# Autodesk Inventor assembly: HopperAssembly_v2
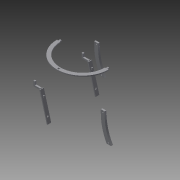
[picture p0: Inventor's stored thumbnail of the model, 180x180]
Saved by Autodesk Inventor 2013 (Build 170138000, 138)
## iProperties
Created: 2013-01-17
Part Number: HopperAssembly_v2
Document SubType Name: Assembly
Designer: twsass
Author: twsass
## Documents named in this file (5)
- E:\Robotics\Hopper\HopperAssembly_v2.iam
- E:\Robotics\Hopper\AttachmentPlateHopper_v2.ipt
- E:\Robotics\Hopper\HopperFrontSupport_v1.ipt
- E:\Robotics\Hopper\HopperSupportRod_v1.ipt
- E:\Robotics\Hopper\TopfemaleHoopSection_v1.ipt
## Components (7 placed, 4 different names)
1. AttachmentPlateHopper_v2:1 — Mate:4, Mate:5, Mate:6
2. AttachmentPlateHopper_v2:2 — Mate:1, Mate:2, Mate:3
3. HopperFrontSupport_v1:1
4. HopperFrontSupport_v1:2
5. HopperSupportRod_v1:1 — Mate:4, Mate:5, Mate:6, Mate:7, Mate:8, Flush:1, Flush:2
6. HopperSupportRod_v1:2 — Mate:1, Mate:2, Mate:3, Mate:7, Mate:8, Flush:1, Flush:2
7. TopfemaleHoopSection_v1:1
## Relationships (10: Mate 8, Flush 2)
- Mate:1: AttachmentPlateHopper_v2:2 ↔ HopperSupportRod_v1:2
- Mate:2: AttachmentPlateHopper_v2:2 ↔ HopperSupportRod_v1:2
- Mate:3: AttachmentPlateHopper_v2:2 ↔ HopperSupportRod_v1:2
- Mate:4: AttachmentPlateHopper_v2:1 ↔ HopperSupportRod_v1:1
- Mate:5: AttachmentPlateHopper_v2:1 ↔ HopperSupportRod_v1:1
- Mate:6: AttachmentPlateHopper_v2:1 ↔ HopperSupportRod_v1:1
- Mate:7 (292.1 mm): HopperSupportRod_v1:1 ↔ HopperSupportRod_v1:2
- Mate:8 (292.1 mm): HopperSupportRod_v1:1 ↔ HopperSupportRod_v1:2
- Flush:1: HopperSupportRod_v1:1 ↔ HopperSupportRod_v1:2
- Flush:2: HopperSupportRod_v1:1 ↔ HopperSupportRod_v1:2
